# Autodesk Inventor assembly: 스위치 조립품
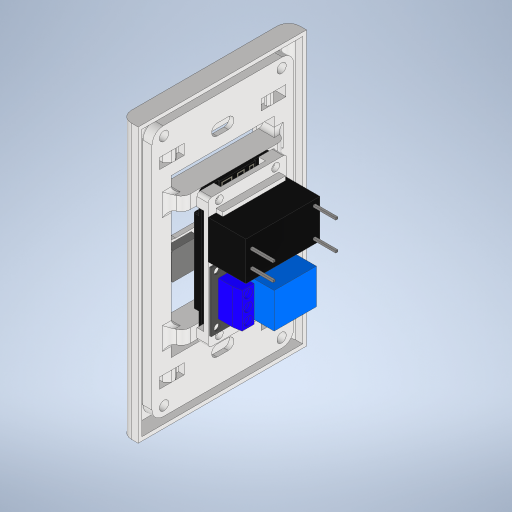
[picture p0: Inventor's stored thumbnail of the model, 512x512]
Saved by Autodesk Inventor 2023 (Build 270158000, 158)
## iProperties
Created: 2022-06-24
Part Number: 스위치 조립품
Document SubType Name: Assembly
Designer: user
Author: user
## Documents named in this file (8)
- C:\Users\user\Desktop\PAI\스마트홈\IOT부품\조명 스위치\스위치 조립품.iam
- C:\Users\user\Desktop\PAI\스마트홈\IOT부품\조명 스위치\조명 케이스.ipt
- C:\Users\user\Desktop\PAI\스마트홈\IOT부품\조명 스위치\스위치 커버.ipt
- C:\Users\user\Desktop\PAI\스마트홈\범용 부품\esp32f.ipt
- C:\Users\user\Desktop\PAI\스마트홈\범용 부품\텍트 스위치.ipt
- C:\Users\user\Desktop\PAI\스마트홈\범용 부품\GMS0205.ipt
- C:\Users\user\Desktop\PAI\스마트홈\범용 부품\릴레이모듈.ipt
- C:\Users\user\Desktop\PAI\스마트홈\IOT부품\조명 스위치\와이파이 모듈 커버.ipt
## Components (8 placed, 7 different names)
1. 조명 케이스:1 — 메이트:1, 메이트:2, 메이트:3, 회전:1, 회전:2, 삽입:1, 삽입:2
2. 스위치 커버:1 — 메이트:1, 메이트:2, 메이트:3
3. esp32f:1 — 삽입:1, 삽입:2, 삽입:3, 삽입:4
4. 텍트 스위치:1 — 회전:2
5. 텍트 스위치:2 — 회전:1
6. GMS0205:1 — 메이트:4, 메이트:7
7. 릴레이모듈:1 — 메이트:6
8. 와이파이 모듈 커버:1 — 삽입:3, 삽입:4, 메이트:4, 메이트:6, 메이트:7
## Relationships (12: Mate 6, Insert 4, RevoluteJoint 2)
- 메이트:1 [Mate]: 조명 케이스:1 ↔ 스위치 커버:1
- 메이트:2 [Mate]: 조명 케이스:1 ↔ 스위치 커버:1
- 메이트:3 [Mate]: 조명 케이스:1 ↔ 스위치 커버:1
- 회전:1 [RevoluteJoint]: 조명 케이스:1 ↔ 텍트 스위치:2
- 회전:2 [RevoluteJoint]: 조명 케이스:1 ↔ 텍트 스위치:1
- 삽입:1 [Insert]: 조명 케이스:1 ↔ esp32f:1
- 삽입:2 [Insert]: 조명 케이스:1 ↔ esp32f:1
- 삽입:3 [Insert]: esp32f:1 ↔ 와이파이 모듈 커버:1
- 삽입:4 [Insert]: esp32f:1 ↔ 와이파이 모듈 커버:1
- 메이트:4 [Mate]: GMS0205:1 ↔ 와이파이 모듈 커버:1
- 메이트:6 [Mate]: 릴레이모듈:1 ↔ 와이파이 모듈 커버:1
- 메이트:7 [Mate]: GMS0205:1 ↔ 와이파이 모듈 커버:1
